# Autodesk Inventor assembly: Llantas
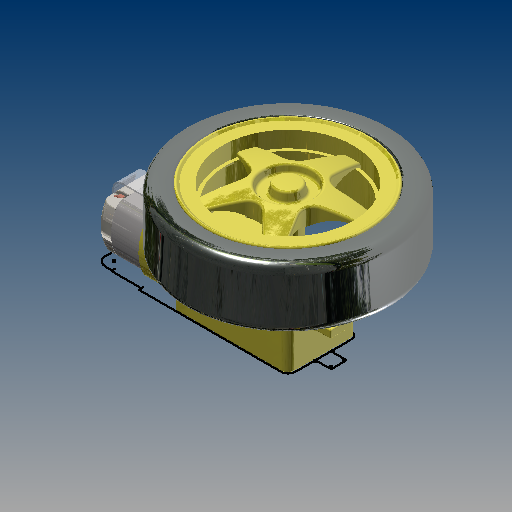
[picture p0: Inventor's stored thumbnail of the model, 512x512]
Saved by Autodesk Inventor 2017 (Build 210142000, 142)
## iProperties
Created: 2017-11-01
Part Number: Llantas
Document SubType Name: Assembly
Designer: Carolina Lema
Author: Carolina Lema
## Documents named in this file (3)
- C:\Users\Carolina Lema\Desktop\ARISE\Teresa Valse\Inventor V2\Llantas.iam
- C:\Users\Carolina Lema\Desktop\ARISE\Teresa Valse\Inventor V2\Moto Reductor 01.ipt
- C:\Users\Carolina Lema\Desktop\ARISE\Teresa Valse\Inventor V2\Rueda 01.ipt
## Components (2 placed, 2 different names)
1. Moto Reductor 01:1 — Mate:1, Mate:2, Tangent:1
2. Rueda 01:1 — Mate:1, Mate:2, Tangent:1
## Relationships (3: Mate 2, Tangent 1)
- Mate:1: Moto Reductor 01:1 ↔ Rueda 01:1
- Mate:2: Moto Reductor 01:1 ↔ Rueda 01:1
- Tangent:1: Moto Reductor 01:1 ↔ Rueda 01:1
